# Autodesk Inventor assembly: Assembly ebeam heater CP V1
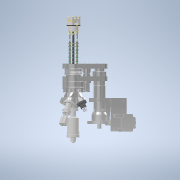
[picture p0: Inventor's stored thumbnail of the model, 180x180]
Saved by Autodesk Inventor 2020 (Build 240168000, 168)
## iProperties
Created: 2019-05-26
Part Number: Assembly ebeam heater CP V1
Document SubType Name: Assembly
Designer: isadmin
Mass: 1360.95 g
Surface Area: 5412.04 cm^2
Volume: 1345.69 cm^3
Density: 1.01134 g/cm^3
Author: isadmin
## Documents named in this file (28)
- C:\Users\ColinP\Documents\Inventor\ebeamheaterv2\Assembly ebeam heater CP V2.iam
- Assembly ebeam heater IS v0.iam
- C:\Users\ColinP\Documents\Inventor\ebeamheaterv2\block.ipt
- C:\Users\ColinP\Documents\Inventor\ebeamheaterv2\Shutter.ipt
- C:\Users\ColinP\Documents\Inventor\ebeamheaterv2\ceramic washer.ipt
- C:\Users\ColinP\Documents\Inventor\ebeamheaterv2\Shielding.ipt
- C:\Users\ColinP\Documents\Inventor\ebeamheaterv2\Bullet_v2_SiliconeSample.ipt
- C:\Users\ColinP\Documents\Inventor\ebeamheaterv2\Bullet_v2_SiliconeSample_TopPart.ipt
- C:\Users\ColinP\Documents\Inventor\ebeamheaterv2\670000.ipt
- C:\Users\ColinP\Documents\Inventor\ebeamheaterv2\MCF275-FlgMplxr-Cr1A5_(53-321020-A).ipt
- C:\Users\ColinP\Documents\Inventor\ebeamheaterv2\665501.ipt
- C:\Users\ColinP\Documents\Inventor\ebeamheaterv2\rotatable rod table.ipt
- C:\Users\ColinP\Documents\Inventor\ebeamheaterv2\updated table+legs.iam
- C:\Users\ColinP\Documents\Inventor\ebeamheaterv2\square eyelet.ipt
- C:\Users\ColinP\Documents\Inventor\ebeamheaterv2\buffer.ipt
- C:\Users\ColinP\Documents\Inventor\ebeamheaterv2\rotaryconnector.ipt
- C:\Users\ColinP\Documents\Inventor\ebeamheaterv2\140007.ipt
- C:\Users\ColinP\Documents\Inventor\ebeamheaterv2\bolt.ipt
- C:\Users\ColinP\Documents\Inventor\Content Center Files\R2020\en-US\ISO 4029\ISO 4029 - M2 x 2 - ISO.ipt
- C:\Users\ColinP\Documents\Inventor\ebeamheaterv2\9312007.iam
- C:\Users\ColinP\Documents\Inventor\ebeamheaterv2\eft0181032.ipt
- C:\Users\ColinP\Documents\Inventor\ebeamheaterv2\filwasher.ipt
- C:\Users\ColinP\Documents\Inventor\ebeamheaterv2\filament.ipt
- C:\Users\ColinP\Documents\Inventor\ebeamheaterv2\fileholddub.ipt
- C:\Users\ColinP\Documents\Inventor\ebeamheaterv2\450000.iam
- C:\Users\ColinP\Documents\Inventor\Content Center Files\R2020\en-US\ISO 4032(2)\ISO 4032 - M3.5 - ISO.ipt
- C:\Users\ColinP\Documents\Inventor\Content Center Files\R2020\en-US\ISO 4032(2)\ISO 4032 - M3 - ISO.ipt
- C:\Users\ColinP\Documents\Inventor\Content Center Files\R2020\en-US\ISO 4017(1)\ISO 4017 - M3 x 6 - ISO.ipt
## Components (158 placed, 26 different names)
1. rotatable rod table:1 — Insert:171, Insert:175, Insert:181, Insert:255, Insert:256, Insert:262, Insert:263, Insert:264, Rigid:20, Insert:266, Insert:268, Insert:269, Insert:270
2. block for bullet:1
3. Shutter:1
4. ceramic washer:1
5. ceramic washer:2
6. ceramic washer:3
7. ceramic washer:4
8. Shielding:1
9. ceramic washer:5
10. ceramic washer:6
11. ceramic washer:7
12. ceramic washer:8
13. Bullet_v2_SiliconeSample:1
14. Bullet_v2_SiliconeSample_TopPart:1
15. rotation_670000:1 — Rotational:3, Rigid:20
16. MCF275-FlgMplxr-Cr1A5_(53-321020-A):1 — Rotational:3, Rigid:5, Rotational:5, Rotational:6, Rotational:10, Rigid:19
17. zstage_665501:1 — Rigid:8, Insert:137, Insert:138, Insert:139, Insert:140, Insert:141, Insert:142
18. 140007:1 — Rigid:5, Rigid:8, Insert:131, Insert:132, Insert:133, Insert:134, Insert:135, Insert:136
19. buffer:5 — Insert:171
20. square eyelet:27 — Insert:206
21. square eyelet:28 — Insert:203, Insert:204
22. square eyelet:29 — Insert:202, Insert:205
23. rotaryconnector:2 — Insert:149, Insert:150, Insert:151, Insert:152
24. square eyelet:49 — Insert:134, Mate:313
25. square eyelet:50 — Insert:135, Mate:311
26. square eyelet:51 — Insert:133, Mate:305
27. square eyelet:52 — Insert:131, Mate:309
28. square eyelet:53 — Insert:132, Mate:307
29. square eyelet:54 — Insert:136, Mate:295, Mate:315
30. bolt:1 — Insert:142
31. bolt:2 — Insert:138
32. bolt:3 — Insert:140
33. bolt:4 — Insert:139
34. bolt:5 — Insert:141
35. bolt:6 — Insert:137
36. buffer:10 — Insert:175
37. square eyelet:55 — Insert:197, Mate:177
38. square eyelet:56 — Insert:199, Insert:200
39. square eyelet:57 — Insert:198, Mate:175
40. 9312007:1 [sub-assembly] — Rotational:5
41. eft0181032:1 — Rotational:6
42. fileholddub:1 — Rigid:17, Rotational:9, Insert:267, Angle:2, Mate:349, Mate:351
43. filwasher:5 — Rotational:9, Mate:343, Mate:350
44. filwasher:6 — Rigid:17, Mate:286, Mate:352
45. buffer:11 — Insert:178, Insert:179, Insert:180, Insert:181
46. square eyelet:67 — Insert:178, Mate:169, Mate:171
47. square eyelet:68 — Insert:179, Mate:167, Mate:173
48. square eyelet:69 — Insert:180, Mate:165, Insert:196
49. ISO 4029 M2 x 2:1 — Insert:152
50. ISO 4029 M2 x 2:2 — Insert:150
51. ISO 4029 M2 x 2:3 — Insert:151
52. ISO 4029 M2 x 2:4 — Insert:149
53. 450000:1 [sub-assembly] — Rigid:19
54. 450000:2 [sub-assembly] — Rotational:10
55. ISO 4032 M3.5:1 — Mate:165
56. ISO 4032 M3.5:2 — Mate:167
57. ISO 4032 M3.5:3 — Mate:169
58. ISO 4032 M3.5:4 — Mate:171
59. ISO 4032 M3.5:5 — Mate:173
60. ISO 4032 M3:1 — Insert:196
61. ISO 4032 M3:2 — Insert:197
62. ISO 4032 M3:3 — Insert:198
63. ISO 4032 M3:4 — Insert:199
64. ISO 4032 M3:5 — Insert:200
65. ISO 4032 M3.5:6 — Mate:175
66. ISO 4032 M3.5:7 — Mate:177, Insert:201
67. ISO 4032 M3.5:8 — Insert:201
68. ISO 4032 M3:6 — Insert:202
69. ISO 4032 M3:7 — Insert:203
70. ISO 4032 M3:8 — Insert:204
71. ISO 4032 M3:9 — Insert:205
72. ISO 4032 M3:10 — Insert:206
73. buffer:14 — Insert:255
74. square eyelet:76 — Mate:199, Mate:209, Mate:297
75. square eyelet:77 — Mate:203, Mate:207
76. square eyelet:78 — Mate:201, Mate:205
77. buffer:15 — Insert:263
78. square eyelet:79 — Mate:237, Mate:241, Mate:300
79. square eyelet:80 — Mate:235, Mate:245
80. square eyelet:81 — Mate:239, Mate:243
81. buffer:16 — Insert:264
82. square eyelet:82 — Mate:211, Mate:217, Mate:298
83. square eyelet:83 — Mate:215, Mate:221
84. square eyelet:84 — Mate:213, Mate:219
85. buffer:17 — Insert:269
86. square eyelet:85 — Mate:319, Mate:325
87. square eyelet:86 — Mate:301, Mate:317, Mate:323
88. square eyelet:87 — Mate:321, Mate:337
89. buffer:18 — Insert:270
90. square eyelet:88 — Mate:302, Mate:327, Mate:331
91. square eyelet:89 — Mate:329, Mate:333
92. square eyelet:90 — Mate:335, Mate:339
93. buffer:19 — Insert:256
94. square eyelet:91 — Mate:271, Mate:279, Mate:303, Mate:341
95. square eyelet:92 — Mate:275, Mate:277
96. square eyelet:93 — Mate:273, Mate:281
97. buffer:20 — Insert:262
98. square eyelet:94 — Mate:225, Mate:231, Mate:299
99. square eyelet:95 — Mate:223, Mate:233
100. square eyelet:96 — Mate:227, Mate:229
101. ISO 4032 M3.5:15 — Mate:199
102. ISO 4032 M3.5:16 — Mate:201
103. ISO 4032 M3.5:17 — Mate:203
104. ISO 4032 M3.5:18 — Mate:205
105. ISO 4032 M3.5:19 — Mate:207
106. ISO 4032 M3.5:20 — Mate:209
107. ISO 4032 M3.5:21 — Mate:211
108. ISO 4032 M3.5:22 — Mate:213
109. ISO 4032 M3.5:23 — Mate:215
110. ISO 4032 M3.5:24 — Mate:217
111. ISO 4032 M3.5:25 — Mate:219
112. ISO 4032 M3.5:26 — Mate:221
113. ISO 4032 M3.5:27 — Mate:223
114. ISO 4032 M3.5:28 — Mate:225
115. ISO 4032 M3.5:29 — Mate:227
116. ISO 4032 M3.5:30 — Mate:229
117. ISO 4032 M3.5:31 — Mate:231
118. ISO 4032 M3.5:32 — Mate:233
119. ISO 4032 M3.5:33 — Mate:235
120. ISO 4032 M3.5:34 — Mate:237
121. ISO 4032 M3.5:35 — Mate:239
122. ISO 4032 M3.5:36 — Mate:241
123. ISO 4032 M3.5:37 — Mate:243
124. ISO 4032 M3.5:38 — Mate:245
125. ISO 4032 M3.5:51 — Mate:271
126. ISO 4032 M3.5:52 — Mate:273
127. ISO 4032 M3.5:53 — Mate:275
128. ISO 4032 M3.5:54 — Mate:277
129. ISO 4032 M3.5:55 — Mate:279, Mate:291
130. ISO 4032 M3.5:56 — Mate:281
131. updated table+legs:2 [sub-assembly] — Insert:266, Insert:267, Angle:2, Rigid:21, Rigid:22, Mate:288, Mate:291, Insert:268, Mate:295, Mate:297, Mate:298, Mate:299, Mate:300, Mate:301, Mate:302, Mate:303, Mate:304, Mate:306, Mate:308, Mate:310, Mate:312, Mate:314, Mate:316, Mate:318, Mate:320, Mate:322, Mate:324, Mate:326, Mate:328, Mate:330, Mate:332, Mate:334, Mate:336, Mate:338, Mate:340, Mate:344, Mate:345, Mate:347
132. filwasher:7 — Rigid:22, Mate:285, Mate:348
133. filwasher:8 — Rigid:21, Mate:342, Mate:346
134. filament:2 — Mate:285, Mate:286, Mate:288
135. ISO 4032 M3.5:57 — Mate:304, Mate:305
136. ISO 4032 M3.5:58 — Mate:306, Mate:307
137. ISO 4032 M3.5:59 — Mate:308, Mate:309
138. ISO 4032 M3:11 — Mate:310, Mate:311
139. ISO 4032 M3:12 — Mate:312, Mate:313
140. ISO 4032 M3:13 — Mate:314, Mate:315
141. ISO 4032 M3.5:60 — Mate:316, Mate:317
142. ISO 4032 M3.5:61 — Mate:318, Mate:319
143. ISO 4032 M3.5:62 — Mate:320, Mate:321
144. ISO 4032 M3.5:63 — Mate:322, Mate:323
145. ISO 4032 M3.5:64 — Mate:324, Mate:325
146. ISO 4032 M3.5:65 — Mate:326, Mate:327
147. ISO 4032 M3.5:66 — Mate:328, Mate:329
148. ISO 4032 M3.5:67 — Mate:330, Mate:331
149. ISO 4032 M3.5:68 — Mate:332, Mate:333
150. ISO 4032 M3.5:69 — Mate:334, Mate:335
151. ISO 4032 M3.5:70 — Mate:336, Mate:337
152. ISO 4032 M3.5:71 — Mate:338, Mate:339
153. ISO 4032 M3.5:72 — Mate:340, Mate:341
154. filament:3 — Mate:342, Mate:343, Mate:344
155. ISO 4017 M3 x 6:1 — Mate:345, Mate:346
156. ISO 4017 M3 x 6:2 — Mate:347, Mate:348
157. ISO 4017 M3 x 6:3 — Mate:349, Mate:350
158. ISO 4017 M3 x 6:4 — Mate:351, Mate:352
## Relationships (208: Mate 120, Insert 73, WeldJoint 7, RevoluteJoint 5, Flush 2, Angle 1)
- [Mate]: block for bullet:1 ↔ Shutter:1
- [Mate]: block for bullet:1 ↔ Shutter:1
- [Mate]: block for bullet:1 ↔ Shutter:1
- [Mate]: block for bullet:1 ↔ ceramic washer:2
- [Mate]: block for bullet:1 ↔ ceramic washer:2
- [Mate]: block for bullet:1 ↔ ceramic washer:1
- [Mate]: block for bullet:1 ↔ ceramic washer:1
- [Mate]: block for bullet:1 ↔ ceramic washer:4
- [Mate]: block for bullet:1 ↔ ceramic washer:4
- [Mate]: block for bullet:1 ↔ ceramic washer:3
- [Mate]: block for bullet:1 ↔ ceramic washer:3
- [Mate]: ceramic washer:1 ↔ Shielding:1
- [Flush]: block for bullet:1 ↔ Shielding:1
- [Flush]: block for bullet:1 ↔ Shielding:1
- [Mate]: block for bullet:1 ↔ ceramic washer:5
- [Mate]: block for bullet:1 ↔ ceramic washer:5
- [Mate]: block for bullet:1 ↔ ceramic washer:6
- [Mate]: block for bullet:1 ↔ ceramic washer:6
- [Mate]: block for bullet:1 ↔ ceramic washer:7
- [Mate]: block for bullet:1 ↔ ceramic washer:7
- [Mate]: block for bullet:1 ↔ ceramic washer:8
- [Mate]: block for bullet:1 ↔ ceramic washer:8
- [Mate] (0.0254 mm): Bullet_v2_SiliconeSample:1 ↔ Bullet_v2_SiliconeSample_TopPart:1
- [Mate]: Bullet_v2_SiliconeSample:1 ↔ Bullet_v2_SiliconeSample_TopPart:1
- [Insert]: block for bullet:1 ↔ Bullet_v2_SiliconeSample:1
- [Insert]: rotatable rod table:1 ↔ block for bullet:1
- [Insert]: rotatable rod table:1 ↔ block for bullet:1
- [Insert]: buffer:5 ↔ square eyelet:28
- [Insert]: buffer:5 ↔ square eyelet:27
- [Insert]: buffer:5 ↔ square eyelet:29
- Rotational:3 [RevoluteJoint]: rotation_670000:1 ↔ MCF275-FlgMplxr-Cr1A5_(53-321020-A):1
- Rigid:5 [WeldJoint]: MCF275-FlgMplxr-Cr1A5_(53-321020-A):1 ↔ 140007:1
- Rigid:8 [WeldJoint]: zstage_665501:1 ↔ 140007:1
- Insert:131: 140007:1 ↔ square eyelet:52
- Insert:132: 140007:1 ↔ square eyelet:53
- Insert:133: 140007:1 ↔ square eyelet:51
- Insert:134: 140007:1 ↔ square eyelet:49
- Insert:135: 140007:1 ↔ square eyelet:50
- Insert:136: 140007:1 ↔ square eyelet:54
- Insert:137: zstage_665501:1 ↔ bolt:6
- Insert:138: zstage_665501:1 ↔ bolt:2
- Insert:139: zstage_665501:1 ↔ bolt:4
- Insert:140: zstage_665501:1 ↔ bolt:3
- Insert:141: zstage_665501:1 ↔ bolt:5
- Insert:142: zstage_665501:1 ↔ bolt:1
- [Insert]: buffer:10 ↔ square eyelet:56
- [Insert]: buffer:10 ↔ square eyelet:55
- [Insert]: buffer:10 ↔ square eyelet:57
- Insert:149: rotaryconnector:2 ↔ ISO 4029 M2 x 2:4
- Insert:150: rotaryconnector:2 ↔ ISO 4029 M2 x 2:2
- Insert:151: rotaryconnector:2 ↔ ISO 4029 M2 x 2:3
- Insert:152: rotaryconnector:2 ↔ ISO 4029 M2 x 2:1
- Rotational:5 [RevoluteJoint]: MCF275-FlgMplxr-Cr1A5_(53-321020-A):1 ↔ 9312007:1
- Rotational:6 [RevoluteJoint]: MCF275-FlgMplxr-Cr1A5_(53-321020-A):1 ↔ eft0181032:1
- Rigid:17 [WeldJoint]: fileholddub:1 ↔ filwasher:6
- Rotational:9 [RevoluteJoint]: fileholddub:1 ↔ filwasher:5
- Insert:171 (163.83 mm): rotatable rod table:1 ↔ buffer:5
- Insert:175 (152.4 mm): rotatable rod table:1 ↔ buffer:10
- Insert:178: buffer:11 ↔ square eyelet:67
- Insert:179: buffer:11 ↔ square eyelet:68
- Insert:180: buffer:11 ↔ square eyelet:69
- Insert:181 (140.97 mm): rotatable rod table:1 ↔ buffer:11
- Rotational:10 [RevoluteJoint]: MCF275-FlgMplxr-Cr1A5_(53-321020-A):1 ↔ 450000:2
- Rigid:19 [WeldJoint]: MCF275-FlgMplxr-Cr1A5_(53-321020-A):1 ↔ 450000:1
- Mate:165: square eyelet:69 ↔ ISO 4032 M3.5:1
- Mate:167: square eyelet:68 ↔ ISO 4032 M3.5:2
- Mate:169: square eyelet:67 ↔ ISO 4032 M3.5:3
- Mate:171: square eyelet:67 ↔ ISO 4032 M3.5:4
- Mate:173: square eyelet:68 ↔ ISO 4032 M3.5:5
- Insert:196: square eyelet:69 ↔ ISO 4032 M3:1
- Insert:197: square eyelet:55 ↔ ISO 4032 M3:2
- Insert:198: square eyelet:57 ↔ ISO 4032 M3:3
- Insert:199: square eyelet:56 ↔ ISO 4032 M3:4
- Insert:200: square eyelet:56 ↔ ISO 4032 M3:5
- Mate:175: square eyelet:57 ↔ ISO 4032 M3.5:6
- Mate:177: square eyelet:55 ↔ ISO 4032 M3.5:7
- Insert:201: ISO 4032 M3.5:7 ↔ ISO 4032 M3.5:8
- Insert:202: square eyelet:29 ↔ ISO 4032 M3:6
- Insert:203: square eyelet:28 ↔ ISO 4032 M3:7
- Insert:204: square eyelet:28 ↔ ISO 4032 M3:8
- Insert:205: square eyelet:29 ↔ ISO 4032 M3:9
- Insert:206: square eyelet:27 ↔ ISO 4032 M3:10
- [Insert]: buffer:14 ↔ square eyelet:76
- [Insert]: buffer:14 ↔ square eyelet:77
- [Insert]: buffer:14 ↔ square eyelet:78
- [Insert]: buffer:15 ↔ square eyelet:79
- [Insert]: buffer:15 ↔ square eyelet:80
- [Insert]: buffer:15 ↔ square eyelet:81
- [Insert]: buffer:16 ↔ square eyelet:82
- [Insert]: buffer:16 ↔ square eyelet:83
- [Insert]: buffer:16 ↔ square eyelet:84
- [Insert]: buffer:17 ↔ square eyelet:85
- [Insert]: buffer:17 ↔ square eyelet:86
- [Insert]: buffer:17 ↔ square eyelet:87
- [Insert]: buffer:18 ↔ square eyelet:88
- [Insert]: buffer:18 ↔ square eyelet:89
- [Insert]: buffer:18 ↔ square eyelet:90
- [Insert]: buffer:19 ↔ square eyelet:91
- [Insert]: buffer:19 ↔ square eyelet:92
- [Insert]: buffer:19 ↔ square eyelet:93
- Insert:255 (129.54 mm): rotatable rod table:1 ↔ buffer:14
- Insert:256 (55.88 mm): rotatable rod table:1 ↔ buffer:19
- [Insert]: buffer:20 ↔ square eyelet:94
- [Insert]: buffer:20 ↔ square eyelet:95
- [Insert]: buffer:20 ↔ square eyelet:96
- Insert:262 (102.87 mm): rotatable rod table:1 ↔ buffer:20
- Insert:263 (90.17 mm): rotatable rod table:1 ↔ buffer:15
- Mate:199: square eyelet:76 ↔ ISO 4032 M3.5:15
- Mate:201: square eyelet:78 ↔ ISO 4032 M3.5:16
- Mate:203: square eyelet:77 ↔ ISO 4032 M3.5:17
- Mate:205: square eyelet:78 ↔ ISO 4032 M3.5:18
- Mate:207: square eyelet:77 ↔ ISO 4032 M3.5:19
- Mate:209: square eyelet:76 ↔ ISO 4032 M3.5:20
- Insert:264 (114.935 mm): rotatable rod table:1 ↔ buffer:16
- Mate:211: square eyelet:82 ↔ ISO 4032 M3.5:21
- Mate:213: square eyelet:84 ↔ ISO 4032 M3.5:22
- Mate:215: square eyelet:83 ↔ ISO 4032 M3.5:23
- Mate:217: square eyelet:82 ↔ ISO 4032 M3.5:24
- Mate:219: square eyelet:84 ↔ ISO 4032 M3.5:25
- Mate:221: square eyelet:83 ↔ ISO 4032 M3.5:26
- Mate:223: square eyelet:95 ↔ ISO 4032 M3.5:27
- Mate:225: square eyelet:94 ↔ ISO 4032 M3.5:28
- Mate:227: square eyelet:96 ↔ ISO 4032 M3.5:29
- Mate:229: square eyelet:96 ↔ ISO 4032 M3.5:30
- Mate:231: square eyelet:94 ↔ ISO 4032 M3.5:31
- Mate:233: square eyelet:95 ↔ ISO 4032 M3.5:32
- Mate:235: square eyelet:80 ↔ ISO 4032 M3.5:33
- Mate:237: square eyelet:79 ↔ ISO 4032 M3.5:34
- Mate:239: square eyelet:81 ↔ ISO 4032 M3.5:35
- Mate:241: square eyelet:79 ↔ ISO 4032 M3.5:36
- Mate:243: square eyelet:81 ↔ ISO 4032 M3.5:37
- Mate:245: square eyelet:80 ↔ ISO 4032 M3.5:38
- Mate:271: square eyelet:91 ↔ ISO 4032 M3.5:51
- Mate:273: square eyelet:93 ↔ ISO 4032 M3.5:52
- Mate:275: square eyelet:92 ↔ ISO 4032 M3.5:53
- Mate:277: square eyelet:92 ↔ ISO 4032 M3.5:54
- Mate:279: square eyelet:91 ↔ ISO 4032 M3.5:55
- Mate:281: square eyelet:93 ↔ ISO 4032 M3.5:56
- Rigid:20 [WeldJoint]: rotatable rod table:1 ↔ rotation_670000:1
- Insert:266: rotatable rod table:1 ↔ updated table+legs:2
- Insert:267 (-8.89 mm): fileholddub:1 ↔ updated table+legs:2
- Angle:2 (0 deg): fileholddub:1 ↔ updated table+legs:2
- Rigid:21 [WeldJoint]: updated table+legs:2 ↔ filwasher:8
- Rigid:22 [WeldJoint]: updated table+legs:2 ↔ filwasher:7
- Mate:285: filwasher:7 ↔ filament:2
- Mate:286: filwasher:6 ↔ filament:2
- Mate:288: updated table+legs:2 ↔ filament:2
- Mate:291: ISO 4032 M3.5:55 ↔ updated table+legs:2
- Insert:268: rotatable rod table:1 ↔ updated table+legs:2
- Mate:295: square eyelet:54 ↔ updated table+legs:2
- Insert:269 (78.74 mm): rotatable rod table:1 ↔ buffer:17
- Insert:270 (66.675 mm): rotatable rod table:1 ↔ buffer:18
- Mate:297: square eyelet:76 ↔ updated table+legs:2
- Mate:298: square eyelet:82 ↔ updated table+legs:2
- Mate:299: square eyelet:94 ↔ updated table+legs:2
- Mate:300: square eyelet:79 ↔ updated table+legs:2
- Mate:301: square eyelet:86 ↔ updated table+legs:2
- Mate:302: square eyelet:88 ↔ updated table+legs:2
- Mate:303: square eyelet:91 ↔ updated table+legs:2
- Mate:304: updated table+legs:2 ↔ ISO 4032 M3.5:57
- Mate:305: square eyelet:51 ↔ ISO 4032 M3.5:57
- Mate:306: updated table+legs:2 ↔ ISO 4032 M3.5:58
- Mate:307: square eyelet:53 ↔ ISO 4032 M3.5:58
- Mate:308: updated table+legs:2 ↔ ISO 4032 M3.5:59
- Mate:309: square eyelet:52 ↔ ISO 4032 M3.5:59
- Mate:310: updated table+legs:2 ↔ ISO 4032 M3:11
- Mate:311: square eyelet:50 ↔ ISO 4032 M3:11
- Mate:312: updated table+legs:2 ↔ ISO 4032 M3:12
- Mate:313: square eyelet:49 ↔ ISO 4032 M3:12
- Mate:314: updated table+legs:2 ↔ ISO 4032 M3:13
- Mate:315: square eyelet:54 ↔ ISO 4032 M3:13
- Mate:316: updated table+legs:2 ↔ ISO 4032 M3.5:60
- Mate:317: square eyelet:86 ↔ ISO 4032 M3.5:60
- Mate:318: updated table+legs:2 ↔ ISO 4032 M3.5:61
- Mate:319: square eyelet:85 ↔ ISO 4032 M3.5:61
- Mate:320: updated table+legs:2 ↔ ISO 4032 M3.5:62
- Mate:321: square eyelet:87 ↔ ISO 4032 M3.5:62
- Mate:322: updated table+legs:2 ↔ ISO 4032 M3.5:63
- Mate:323: square eyelet:86 ↔ ISO 4032 M3.5:63
- Mate:324: updated table+legs:2 ↔ ISO 4032 M3.5:64
- Mate:325: square eyelet:85 ↔ ISO 4032 M3.5:64
- Mate:326: updated table+legs:2 ↔ ISO 4032 M3.5:65
- Mate:327: square eyelet:88 ↔ ISO 4032 M3.5:65
- Mate:328: updated table+legs:2 ↔ ISO 4032 M3.5:66
- Mate:329: square eyelet:89 ↔ ISO 4032 M3.5:66
- Mate:330: updated table+legs:2 ↔ ISO 4032 M3.5:67
- Mate:331: square eyelet:88 ↔ ISO 4032 M3.5:67
- Mate:332: updated table+legs:2 ↔ ISO 4032 M3.5:68
- Mate:333: square eyelet:89 ↔ ISO 4032 M3.5:68
- Mate:334: updated table+legs:2 ↔ ISO 4032 M3.5:69
- Mate:335: square eyelet:90 ↔ ISO 4032 M3.5:69
- Mate:336: updated table+legs:2 ↔ ISO 4032 M3.5:70
- Mate:337: square eyelet:87 ↔ ISO 4032 M3.5:70
- Mate:338: updated table+legs:2 ↔ ISO 4032 M3.5:71
- Mate:339: square eyelet:90 ↔ ISO 4032 M3.5:71
- Mate:340: updated table+legs:2 ↔ ISO 4032 M3.5:72
- Mate:341: square eyelet:91 ↔ ISO 4032 M3.5:72
- Mate:342: filwasher:8 ↔ filament:3
- Mate:343: filwasher:5 ↔ filament:3
- Mate:344: updated table+legs:2 ↔ filament:3
- Mate:345: updated table+legs:2 ↔ ISO 4017 M3 x 6:1
- Mate:346: filwasher:8 ↔ ISO 4017 M3 x 6:1
- Mate:347: updated table+legs:2 ↔ ISO 4017 M3 x 6:2
- Mate:348: filwasher:7 ↔ ISO 4017 M3 x 6:2
- Mate:349: fileholddub:1 ↔ ISO 4017 M3 x 6:3
- Mate:350: filwasher:5 ↔ ISO 4017 M3 x 6:3
- Mate:351: fileholddub:1 ↔ ISO 4017 M3 x 6:4
- Mate:352: filwasher:6 ↔ ISO 4017 M3 x 6:4
## Named parameters: d75_d58 = 0 mm, d76_d19 = 0 mm, d77_d22_d25 = 0 mm, d78_d23_d26 = 0 mm, d79_d24_d35 = 0 mm, d80_d25_d36 = 0 mm, d81_d26_d37 = 0 mm, d82_d27_d38 = 0 mm, d83_d28_d39 = 0 mm, d84_d29_d40 = 0 mm, d85_d30_d41 = 0 mm, d86_d31_d42 = 0 mm, d87_d43 = 0 mm, d88_d44 = 0 mm, d89_d45 = 0 mm, d90_d46 = 0 mm, d91_d47 = 0 mm, d92_d48 = 0 mm, d93_d49 = 0 mm, d94_d50 = 0 mm, d95_d51 = 0 mm, d96_d52 = 0 mm, d97_d53 = 0 mm, d98_d56_d0 = 0.0254 mm, d99_d57_d1 = 0 mm, d152_d124_d114_d111 = 0 mm, d153_d125_d115_d112 = 0 mm, d154_d126_d116_d113 = 0 mm, d314_d124_d114_d111 = 0 mm, d315_d125_d115_d112 = 0 mm, d316_d126_d116_d113 = 0 mm, d835_d606 = 0 mm, d836_d607 = 0 mm, d837_d608 = 0 mm, d838_d606 = 0 mm, d839_d607 = 0 mm, d840_d608 = 0 mm, d841_d606 = 0 mm, d842_d607 = 0 mm, d843_d608 = 0 mm, d844_d606 = 0 mm, d845_d607 = 0 mm, d846_d608 = 0 mm, d847_d606 = 0 mm, d848_d607 = 0 mm, d849_d608 = 0 mm, d850_d606 = 0 mm, d851_d607 = 0 mm, d852_d608 = 0 mm, d863_d844_d606 = 0 mm, d864_d845_d607 = 0 mm, d865_d846_d608 = 0 mm
